# Autodesk Inventor assembly: Vex Traction Wheel 4x1.5
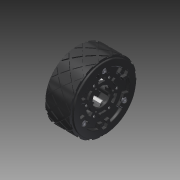
[picture p0: Inventor's stored thumbnail of the model, 180x180]
Saved by Autodesk Inventor 2013 (Build 170138000, 138)
## iProperties
Created: 2012-12-09
Part Number: Vex Traction Wheel 4x1.5
Document SubType Name: Assembly
Designer: Nemo
Author: Nemo
## Documents named in this file (7)
- \\lmss\STUDENTS\Robotics\CAD Files\COTS Parts\Wheels\VexPro Traction Wheels\Vex Traction Wheel 4x1.5.iam
- \\lmss\STUDENTS\Robotics\CAD Files\COTS Parts\Wheels\VexPro Traction Wheels\Components\Traction Tire Body 4in.ipt
- \\lmss\STUDENTS\Robotics\CAD Files\COTS Parts\Wheels\VexPro Traction Wheels\Components\Traction Tire extension 4in.ipt
- \\lmss\STUDENTS\Robotics\CAD Files\COTS Parts\Fasteners\Hex Standoff 8-32 x1250.ipt
- \\lmss\STUDENTS\Robotics\CAD Files\COTS Parts\Wheels\VexPro Traction Wheels\Components\4 Traction Tire - 1.5 Wide.ipt
- \\lmss\STUDENTS\Robotics\CAD Files\COTS Parts\Fasteners\8-32 locknut.ipt
- \\lmss\STUDENTS\Robotics\CAD Files\COTS Parts\Fasteners\8-32 BHCS x1750.ipt
## Components (16 placed, 6 different names)
1. Traction Tire Body 4in:1 — Mate:1, Mate:2, Mate:3, Mate:4, Mate:5, Mate:6, Mate:9, Angle:1, Mate:10, Insert:2, Angle:2
2. Traction Tire Body 4in:2 — Mate:3, Mate:7, Mate:8, Insert:1
3. Traction Tire extension 4in:1 — Mate:4, Mate:5, Mate:6, Flush:1, Mate:7, Mate:8
4. 4 Traction Tire - 1.5 Wide:1 — Mate:11, Mate:12, Mate:13
5. Hex Standoff 8-32 x1250:1 — Mate:9, Angle:1, Mate:10
6. Hex Standoff 8-32 x1250:2
7. Hex Standoff 8-32 x1250:3
8. Hex Standoff 8-32 x1250:4
9. Hex Standoff 8-32 x1250:5
10. Hex Standoff 8-32 x1250:6
11. 8-32 BHCS x1750:1 — Insert:1
12. 8-32 locknut:1 — Insert:2, Angle:2
13. 8-32 BHCS x1750:2
14. 8-32 locknut:2
15. 8-32 BHCS x1750:3
16. 8-32 locknut:3
## Component patterns: (6 elements, first: Hex Standoff 8-32 x1250:1), (3 elements, first: 8-32 BHCS x1750:1 + 8-32 locknut:1)
## Relationships (18: Mate 13, Angle 2, Insert 2, Flush 1)
- Mate:1: Traction Tire Body 4in:1
- Mate:2: Traction Tire Body 4in:1
- Mate:3: Traction Tire Body 4in:1 ↔ Traction Tire Body 4in:2
- Mate:4: Traction Tire Body 4in:1 ↔ Traction Tire extension 4in:1
- Mate:5: Traction Tire Body 4in:1 ↔ Traction Tire extension 4in:1
- Mate:6: Traction Tire Body 4in:1 ↔ Traction Tire extension 4in:1
- Flush:1: Traction Tire extension 4in:1
- Mate:7: Traction Tire Body 4in:2 ↔ Traction Tire extension 4in:1
- Mate:8: Traction Tire Body 4in:2 ↔ Traction Tire extension 4in:1
- Mate:9: Traction Tire Body 4in:1 ↔ Hex Standoff 8-32 x1250:1
- Angle:1 (0 deg): Traction Tire Body 4in:1 ↔ Hex Standoff 8-32 x1250:1
- Mate:10: Traction Tire Body 4in:1 ↔ Hex Standoff 8-32 x1250:1
- Mate:11: 4 Traction Tire - 1.5 Wide:1
- Mate:12: 4 Traction Tire - 1.5 Wide:1
- Mate:13: 4 Traction Tire - 1.5 Wide:1
- Insert:1: Traction Tire Body 4in:2 ↔ 8-32 BHCS x1750:1
- Insert:2: Traction Tire Body 4in:1 ↔ 8-32 locknut:1
- Angle:2 (0 deg): Traction Tire Body 4in:1 ↔ 8-32 locknut:1
